# Autodesk Inventor assembly: BigGear
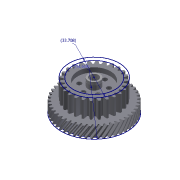
[picture p0: Inventor's stored thumbnail of the model, 180x180]
Saved by Autodesk Inventor 2012 (Build 160160000, 160)
## iProperties
Created: 2017-01-26
Part Number: BigGear
Document SubType Name: Assembly
Designer: omaro
Mass: 114.67 g
Surface Area: 109.53 cm^2
Volume: 15.1388 cm^3
Density: 7.57458 g/cm^3
Author: omaro
## Documents named in this file (5)
- C:\Projects\originalGate\GateProject-master\GateProjectMain\Hardware\Mechanical\BigGear.iam
- C:\Projects\originalGate\GateProject-master\GateProjectMain\Hardware\Mechanical\BigGear\Design Accelerator\Spur Gears3.iam
- C:\Projects\originalGate\GateProject-master\GateProjectMain\Hardware\Mechanical\Assembly1\Design Accelerator\Spur Gears1.iam
- C:\Projects\originalGate\GateProject-master\GateProjectMain\Hardware\Mechanical\Assembly1\Design Accelerator\Spur Gears3.iam
- C:\Projects\originalGate\GateProject-master\GateProjectMain\Hardware\Mechanical\BigGearShaft.ipt
## Components (3 placed, 2 different names)
1. Spur Gears:3 [sub-assembly] — Mate:1, Flush:1, Mate:2
2. Spur Gears:4 [sub-assembly] — Mate:1, Mate:3
3. BigGearShaft:1 — Flush:1, Mate:2, Mate:3
## Relationships (4: Mate 3, Flush 1)
- Mate:1: Spur Gears:3 ↔ Spur Gears:4
- Flush:1: Spur Gears:3 ↔ BigGearShaft:1
- Mate:2: Spur Gears:3 ↔ BigGearShaft:1
- Mate:3: Spur Gears:4 ↔ BigGearShaft:1
